# Autodesk Inventor assembly: Ensemble1
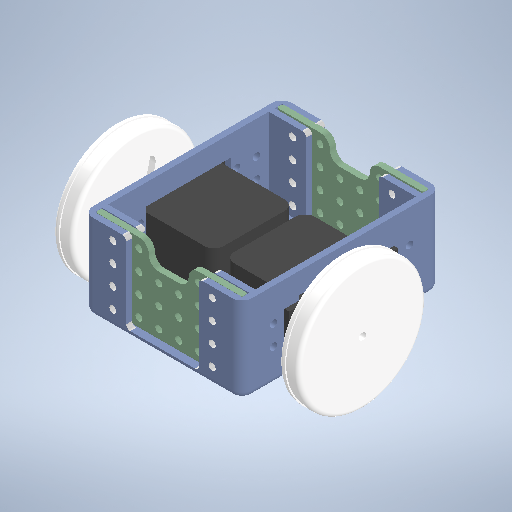
[picture p0: Inventor's stored thumbnail of the model, 512x512]
Saved by Autodesk Inventor 2025 (Build 290162000, 162)
## iProperties
Created: 2024-09-06
Part Number: Ensemble1
Document SubType Name: Assembly
Designer: chass
Author: chass
## Documents named in this file (5)
- C:\Users\chass\Documents\Inventor\Projets\Hackathon\Ensemble1.iam
- C:\Users\chass\Documents\Inventor\Projets\Hackathon\chassis.ipt
- C:\Users\chass\Documents\Inventor\Projets\Hackathon\servomoteur_roues.ipt
- C:\Users\chass\Documents\Inventor\Projets\Hackathon\plaque.ipt
- C:\Users\chass\Documents\Inventor\Projets\Hackathon\roue.ipt
## Components (7 placed, 4 different names)
1. chassis:1 — Placage:1, Placage:2, Placage:3, Placage:4, Placage:5, Placage:6, Placage:16, Placage:17, Placage:18, Placage:19
2. servomoteur_roues:1 — Placage:1, Placage:2, Placage:3, Placage:14, Placage:15
3. servomoteur_roues:2 — Placage:4, Placage:5, Placage:6, Placage:12, Placage:13
4. plaque:1 — Placage:18, Placage:19
5. plaque:2 — Placage:16, Placage:17
6. roue:1 — Placage:12, Placage:13
7. roue:2 — Placage:14, Placage:15
## Relationships (14: Mate 14)
- Placage:1 [Mate]: chassis:1 ↔ servomoteur_roues:1
- Placage:2 [Mate]: chassis:1 ↔ servomoteur_roues:1
- Placage:3 [Mate]: chassis:1 ↔ servomoteur_roues:1
- Placage:4 [Mate]: chassis:1 ↔ servomoteur_roues:2
- Placage:5 [Mate]: chassis:1 ↔ servomoteur_roues:2
- Placage:6 [Mate]: chassis:1 ↔ servomoteur_roues:2
- Placage:12 [Mate]: servomoteur_roues:2 ↔ roue:1
- Placage:13 [Mate]: servomoteur_roues:2 ↔ roue:1
- Placage:14 [Mate]: servomoteur_roues:1 ↔ roue:2
- Placage:15 [Mate]: servomoteur_roues:1 ↔ roue:2
- Placage:16 [Mate]: chassis:1 ↔ plaque:2
- Placage:17 [Mate]: chassis:1 ↔ plaque:2
- Placage:18 [Mate]: chassis:1 ↔ plaque:1
- Placage:19 [Mate]: chassis:1 ↔ plaque:1
